# Autodesk Inventor assembly: MeltyAssembly
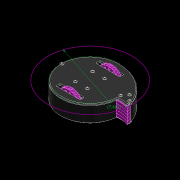
[picture p0: Inventor's stored thumbnail of the model, 180x180]
Saved by Autodesk Inventor 2022 (Build 260153000, 153)
## iProperties
Created: 2022-05-03
Part Number: MeltyAssembly
Document SubType Name: Assembly
Designer: tandu
Mass: 450.028 g
Surface Area: 1390.68 cm^2
Volume: 291.526 cm^3
Author: tandu
## Documents named in this file (8)
- C:\Users\tandu\Documents\GrabCAD\1 Pound Melty\MeltyAssembly.iam
- C:\Users\tandu\Documents\GrabCAD\1 Pound Melty\MeltyBrainChassis.ipt
- C:\Users\tandu\Documents\GrabCAD\1 Pound Melty\BatteryMockup.ipt
- C:\Users\tandu\Documents\GrabCAD\1 Pound Melty\EMax RS2205 v1.ipt
- C:\Users\tandu\Documents\GrabCAD\1 Pound Melty\MeltyBrainTooth.ipt
- C:\Users\tandu\Documents\GrabCAD\1 Pound Melty\SimplerFanWheel_v2.ipt
- C:\Users\tandu\Documents\GrabCAD\1 Pound Melty\TopLid.ipt
- C:\Users\tandu\Documents\GrabCAD\1 Pound Melty\90417A126_Phillips Rounded Head Thread-Forming Screws.ipt
## Components (21 placed, 7 different names)
1. MeltyBrainChassis:1 — Insert:2, Insert:3, Insert:4, Insert:5, Flush:1, Flush:2, Flush:3, Flush:4, Insert:11, Mate:3, Mate:4, Mate:6, Mate:7, Mate:9, Mate:10, Mate:12, Mate:13, Mate:14, Tangent:1, Tangent:2, Angle:1
2. BatteryMockup:1 — Mate:14, Tangent:1, Tangent:2, Angle:1
3. EMax RS2205 v1:1 — Insert:4, Insert:5, Insert:6
4. EMax RS2205 v1:2 — Insert:2, Insert:3, Insert:7
5. SimplerFanWheel_v2:1 — Insert:7
6. SimplerFanWheel_v2:2 — Insert:6
7. TopLid:1 — Flush:3, Flush:4, Insert:8, Insert:9, Insert:10, Insert:12, Insert:13, Insert:14, Insert:15, Insert:16
8. MeltyBrainTooth:2 — Mate:2, Mate:3, Mate:4, Mate:5
9. MeltyBrainTooth:3 — Mate:5, Mate:6, Mate:7, Mate:8
10. MeltyBrainTooth:4 — Mate:8, Mate:9, Mate:10, Mate:11
11. MeltyBrainTooth:5 — Mate:11, Mate:12, Mate:13
12. MeltyBrainTooth:1 — Flush:1, Flush:2, Mate:2
13. 90417A126_Phillips Rounded Head Thread-Forming Screws:1 — Insert:16
14. 90417A126_Phillips Rounded Head Thread-Forming Screws:2 — Insert:15
15. 90417A126_Phillips Rounded Head Thread-Forming Screws:3 — Insert:13
16. 90417A126_Phillips Rounded Head Thread-Forming Screws:4 — Insert:12
17. 90417A126_Phillips Rounded Head Thread-Forming Screws:5 — Insert:14
18. 90417A126_Phillips Rounded Head Thread-Forming Screws:6 — Insert:10
19. 90417A126_Phillips Rounded Head Thread-Forming Screws:7 — Insert:8
20. 90417A126_Phillips Rounded Head Thread-Forming Screws:8 — Insert:9
21. 90417A126_Phillips Rounded Head Thread-Forming Screws:9 — Insert:11
## Relationships (35: Insert 15, Mate 13, Flush 4, Tangent 2, Angle 1)
- Insert:2: MeltyBrainChassis:1 ↔ EMax RS2205 v1:2
- Insert:3: MeltyBrainChassis:1 ↔ EMax RS2205 v1:2
- Insert:4: MeltyBrainChassis:1 ↔ EMax RS2205 v1:1
- Insert:5: MeltyBrainChassis:1 ↔ EMax RS2205 v1:1
- Flush:1: MeltyBrainChassis:1 ↔ MeltyBrainTooth:1
- Flush:2: MeltyBrainChassis:1 ↔ MeltyBrainTooth:1
- Insert:6: EMax RS2205 v1:1 ↔ SimplerFanWheel_v2:2
- Insert:7: EMax RS2205 v1:2 ↔ SimplerFanWheel_v2:1
- Flush:3: MeltyBrainChassis:1 ↔ TopLid:1
- Flush:4: MeltyBrainChassis:1 ↔ TopLid:1
- Insert:8: TopLid:1 ↔ 90417A126_Phillips Rounded Head Thread-Forming Screws:7
- Insert:9: TopLid:1 ↔ 90417A126_Phillips Rounded Head Thread-Forming Screws:8
- Insert:10: TopLid:1 ↔ 90417A126_Phillips Rounded Head Thread-Forming Screws:6
- Insert:11: MeltyBrainChassis:1 ↔ 90417A126_Phillips Rounded Head Thread-Forming Screws:9
- Insert:12: TopLid:1 ↔ 90417A126_Phillips Rounded Head Thread-Forming Screws:4
- Insert:13: TopLid:1 ↔ 90417A126_Phillips Rounded Head Thread-Forming Screws:3
- Insert:14: TopLid:1 ↔ 90417A126_Phillips Rounded Head Thread-Forming Screws:5
- Insert:15: TopLid:1 ↔ 90417A126_Phillips Rounded Head Thread-Forming Screws:2
- Insert:16: TopLid:1 ↔ 90417A126_Phillips Rounded Head Thread-Forming Screws:1
- Mate:2: MeltyBrainTooth:2 ↔ MeltyBrainTooth:1
- Mate:3: MeltyBrainChassis:1 ↔ MeltyBrainTooth:2
- Mate:4: MeltyBrainChassis:1 ↔ MeltyBrainTooth:2
- Mate:5: MeltyBrainTooth:2 ↔ MeltyBrainTooth:3
- Mate:6: MeltyBrainChassis:1 ↔ MeltyBrainTooth:3
- Mate:7: MeltyBrainChassis:1 ↔ MeltyBrainTooth:3
- Mate:8: MeltyBrainTooth:3 ↔ MeltyBrainTooth:4
- Mate:9: MeltyBrainChassis:1 ↔ MeltyBrainTooth:4
- Mate:10: MeltyBrainChassis:1 ↔ MeltyBrainTooth:4
- Mate:11: MeltyBrainTooth:4 ↔ MeltyBrainTooth:5
- Mate:12: MeltyBrainChassis:1 ↔ MeltyBrainTooth:5
- Mate:13: MeltyBrainChassis:1 ↔ MeltyBrainTooth:5
- Mate:14: MeltyBrainChassis:1 ↔ BatteryMockup:1
- Tangent:1: MeltyBrainChassis:1 ↔ BatteryMockup:1
- Tangent:2: MeltyBrainChassis:1 ↔ BatteryMockup:1
- Angle:1 (180 deg): MeltyBrainChassis:1 ↔ BatteryMockup:1
